# Autodesk Inventor assembly: onderpoot
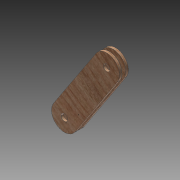
[picture p0: Inventor's stored thumbnail of the model, 180x180]
Saved by Autodesk Inventor 2015 (Build 190159000, 159)
## iProperties
Created: 2016-02-03
Part Number: onderpoot
Document SubType Name: Assembly
Designer: david
Author: david
## Documents named in this file (2)
- Z:\gip\Inventor\generatie 7\Beenen\onderbeen\onderpoot.iam
- Z:\gip\Inventor\generatie 7\Beenen\onderbeen\onderbeen.ipt
## Components (2 placed, 1 different names)
1. onderbeen:1 — Mate:1, Mate:2, Mate:3
2. onderbeen:2 — Mate:1, Mate:2, Mate:3
## Relationships (3: Mate 3)
- Mate:1 (6 mm): onderbeen:1 ↔ onderbeen:2
- Mate:2: onderbeen:1 ↔ onderbeen:2
- Mate:3: onderbeen:1 ↔ onderbeen:2
